# Autodesk Inventor assembly: Main assembly
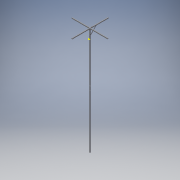
[picture p0: Inventor's stored thumbnail of the model, 180x180]
Saved by Autodesk Inventor 2017 (Build 210142000, 142)
## iProperties
Created: 2018-07-12
Part Number: Main assembly
Document SubType Name: Assembly
Designer: sinner
Author: sinner
## Documents named in this file (10)
- X:\Inventor files\Post\Main assembly.iam
- X:\Inventor files\Post\Lomg horizontal.ipt
- X:\Inventor files\Post\Short horizontal.ipt
- X:\Inventor files\Post\plate 1.ipt
- X:\Inventor files\Post\Vertical.ipt
- X:\Inventor files\Post\Bracket.ipt
- X:\Inventor files\Post\Long support flat.ipt
- X:\Inventor files\Post\Lower Long L.ipt
- X:\Inventor files\Post\Middle short L.ipt
- X:\Inventor files\Post\Upper Long L.ipt
## Components (10 placed, 9 different names)
1. Lomg horizontal:1 — Flush:1, Mate:1, Flush:2, Mate:2, Flush:3, Flush:4, Mate:6, Mate:7, Flush:6, Mate:13
2. Short horizontal:1 — Mate:2, Flush:3, Flush:4, Mate:4, Mate:5, Flush:7, Angle:1
3. Short horizontal:2 — Flush:1, Mate:1, Flush:2, Mate:3
4. plate 1:1 — Mate:3, Mate:4, Mate:5
5. Vertical:1 — Mate:6, Mate:8, Flush:5, Flush:7, Mate:9, Mate:10, Mate:11, Mate:12
6. Bracket:1 — Mate:7, Mate:8, Flush:5, Flush:6
7. Long support flat:1 — Mate:9, Mate:10, Angle:1
8. Lower Long L:1 — Mate:11, Mate:12, Mate:13, Mate:14, Mate:15, Mate:16
9. Middle short L:1 — Mate:14, Mate:15, Mate:16, Mate:17, Mate:18, Mate:19
10. Upper Long L:1 — Mate:17, Mate:18, Mate:19
## Relationships (27: Mate 19, Flush 7, Angle 1)
- Flush:1: Lomg horizontal:1 ↔ Short horizontal:2
- Mate:1: Lomg horizontal:1 ↔ Short horizontal:2
- Flush:2 (596.9 mm): Lomg horizontal:1 ↔ Short horizontal:2
- Mate:2: Lomg horizontal:1 ↔ Short horizontal:1
- Flush:3: Lomg horizontal:1 ↔ Short horizontal:1
- Flush:4 (-596.9 mm): Lomg horizontal:1 ↔ Short horizontal:1
- Mate:3: Short horizontal:2 ↔ plate 1:1
- Mate:4: Short horizontal:1 ↔ plate 1:1
- Mate:5: Short horizontal:1 ↔ plate 1:1
- Mate:6: Lomg horizontal:1 ↔ Vertical:1
- Mate:7: Lomg horizontal:1 ↔ Bracket:1
- Mate:8: Vertical:1 ↔ Bracket:1
- Flush:5: Vertical:1 ↔ Bracket:1
- Flush:6: Lomg horizontal:1 ↔ Bracket:1
- Flush:7: Short horizontal:1 ↔ Vertical:1
- Mate:9: Vertical:1 ↔ Long support flat:1
- Mate:10: Vertical:1 ↔ Long support flat:1
- Angle:1 (135 deg): Short horizontal:1 ↔ Long support flat:1
- Mate:11: Vertical:1 ↔ Lower Long L:1
- Mate:12: Vertical:1 ↔ Lower Long L:1
- Mate:13: Lomg horizontal:1 ↔ Lower Long L:1
- Mate:14: Lower Long L:1 ↔ Middle short L:1
- Mate:15: Lower Long L:1 ↔ Middle short L:1
- Mate:16: Lower Long L:1 ↔ Middle short L:1
- Mate:17: Middle short L:1 ↔ Upper Long L:1
- Mate:18: Middle short L:1 ↔ Upper Long L:1
- Mate:19: Middle short L:1 ↔ Upper Long L:1
